# Autodesk Inventor assembly: SPST-NO Verde
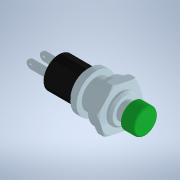
[picture p0: Inventor's stored thumbnail of the model, 180x180]
Saved by Autodesk Inventor 2020.1 (Build 241239000, 239)
## iProperties
Created: 2012-05-21
Part Number: SPST-NO Verde
Document SubType Name: Assembly
Designer: Daniel
Sending System: Autodesk Inventor 2008
Preprocessor: Autodesk Inventor 2008
Title: D:\0 - Biblioteca Inventor\Componentes Electricos\Interruptores\Interruptor Normalmente Aberto 2 Pinos na Base\SPST-NO.stp
Author: jm
## Documents named in this file (4)
- F:\Proyectos\Dog Feeder\Solido\Circuito Electrico\PushButton\SPST-NO Verde.iam
- F:\Proyectos\Dog Feeder\Solido\Circuito Electrico\PushButton\SPST-NO_3.ipt
- F:\Proyectos\Dog Feeder\Solido\Circuito Electrico\PushButton\SPST-NO_2.ipt
- F:\Proyectos\Dog Feeder\Solido\Circuito Electrico\PushButton\SPST-NO_1 Verde.ipt
## Components (3 placed, 3 different names)
1. SPST-NO_1:1 — Mate:1, Mate:2, Mate:3
2. SPST-NO_3:1 — Mate:1, Mate:3, Mate:4
3. SPST-NO_2:1 — Mate:2, Mate:4
## Relationships (4: Mate 4)
- Mate:1: SPST-NO_1:1 ↔ SPST-NO_3:1
- Mate:2: SPST-NO_1:1 ↔ SPST-NO_2:1
- Mate:3 (3 mm): SPST-NO_1:1 ↔ SPST-NO_3:1
- Mate:4: SPST-NO_3:1 ↔ SPST-NO_2:1
